# Autodesk Inventor assembly: luz de freio m
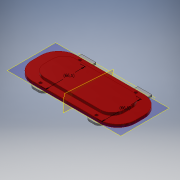
[picture p0: Inventor's stored thumbnail of the model, 180x180]
Saved by Autodesk Inventor 2019 (Build 230136000, 136)
## iProperties
Created: 2020-06-06
Part Number: luz de freio m
Material: Genérico
Document SubType Name: Assembly
Designer: eliane
Author: eliane
## Documents named in this file (3)
- G:\Meu Drive\Projetos\Projeto 2020 2021\Eletrônica 2020-2021\Projeção mecânica\Luz de Freio\luz de freio m.iam
- G:\Meu Drive\Projetos\Projeto 2020 2021\Eletrônica 2020-2021\Projeção mecânica\Luz de Freio\luz de freio.ipt
- G:\Meu Drive\Projetos\Projeto 2020 2021\Eletrônica 2020-2021\Projeção mecânica\Luz de Freio\Fixação luz de freio.ipt
## Components (3 placed, 2 different names)
1. luz de freio:1 — Flush:1, Flush:2, Flush:3, Mate:6, Mate:7, Mate:8, Mate:9, Mate:10, Mate:11, Mate:12, Mate:13, Mate:14, Mate:15, Mate:16, Mate:17
2. Fixação luz de freio:1 — Mate:6, Mate:9, Mate:11, Mate:18
3. Fixação luz de freio:2 — Mate:7, Mate:8, Mate:10, Mate:19
## Relationships (17: Mate 14, Flush 3)
- Flush:1: luz de freio:1
- Flush:2: luz de freio:1
- Flush:3: luz de freio:1
- Mate:6: luz de freio:1 ↔ Fixação luz de freio:1
- Mate:7: luz de freio:1 ↔ Fixação luz de freio:2
- Mate:8: luz de freio:1 ↔ Fixação luz de freio:2
- Mate:9: luz de freio:1 ↔ Fixação luz de freio:1
- Mate:10: luz de freio:1 ↔ Fixação luz de freio:2
- Mate:11: luz de freio:1 ↔ Fixação luz de freio:1
- Mate:12: luz de freio:1
- Mate:13: luz de freio:1
- Mate:14: luz de freio:1
- Mate:15: luz de freio:1
- Mate:16: luz de freio:1
- Mate:17: luz de freio:1
- Mate:18: Fixação luz de freio:1
- Mate:19: Fixação luz de freio:2
